# Autodesk Inventor assembly: AXp4p
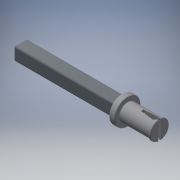
[picture p0: Inventor's stored thumbnail of the model, 180x180]
Saved by Autodesk Inventor 2019.3 (Build 233278000, 278)
## iProperties
Created: 2019-02-08
Part Number: AXp4p
Document SubType Name: Assembly
Designer: Varga Daniel
Author: Varga Daniel
## Documents named in this file (6)
- C:\!_Dani\!_cloud\OneDrive\!_munka\Revolution\RevvyDemoKit\Structural parts\Axles\AXp3+p\AXp4p.iam
- C:\!_Dani\!_cloud\OneDrive\!_munka\Revolution\RevvyDemoKit\Structural parts\Connetor Pins\Connector_pin_collar.ipt
- C:\!_Dani\!_cloud\OneDrive\!_munka\Revolution\RevvyDemoKit\Structural parts\Connetor Pins\Connector_pin_stick.ipt
- C:\!_Dani\!_cloud\OneDrive\!_munka\Revolution\RevvyDemoKit\Structural parts\Axles\One_sided_axle_base.ipt
- C:\!_Dani\!_cloud\OneDrive\!_munka\Revolution\RevvyDemoKit\Structural parts\Axles\AXp3+p.iam
- C:\!_Dani\!_cloud\OneDrive\!_munka\Revolution\RevvyDemoKit\Structural parts\Axles\One_sided_axle_base\One_sided_axle_base-03.ipt
## Components (4 placed, 3 different names)
1. Connector_pin_collar:1 — Mate:1, Mate:2, Mate:3, Mate:4, Mate:5
2. Connector_pin_stick:1 — Mate:1, Mate:2, Angle:1
3. Connector_pin_collar:2 — Mate:3, Mate:4, Mate:6
4. One_sided_axle_base-03:1 — Mate:5, Mate:6, Angle:1
## Relationships (7: Mate 6, Angle 1)
- Mate:1: Connector_pin_collar:1 ↔ Connector_pin_stick:1
- Mate:2: Connector_pin_collar:1 ↔ Connector_pin_stick:1
- Mate:3: Connector_pin_collar:1 ↔ Connector_pin_collar:2
- Mate:4: Connector_pin_collar:1 ↔ Connector_pin_collar:2
- Mate:5: Connector_pin_collar:1 ↔ One_sided_axle_base-03:1
- Mate:6: Connector_pin_collar:2 ↔ One_sided_axle_base-03:1
- Angle:1 (0 deg): Connector_pin_stick:1 ↔ One_sided_axle_base-03:1
